# Autodesk Inventor assembly: Protochip
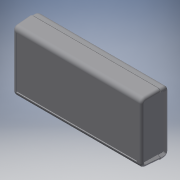
[picture p0: Inventor's stored thumbnail of the model, 180x180]
Saved by Autodesk Inventor 2016 (Build 200138000, 138)
## iProperties
Created: 2011-06-17
Part Number: Protochip
Document SubType Name: Assembly
Designer: David
Title: E:\Eng\Customer Service\Drawings\1593\STEP\1593Y\1593Y Assembly.stp
Author: lwalsh
Sending System: Autodesk Inventor 2011
Preprocessor: Autodesk Inventor 2011
## Documents named in this file (6)
- C:\Users\David\Documents\GitHub\protochip\casing\Protochip.iam
- C:\Users\David\Downloads\1593Y\1593Y Bottom.ipt
- C:\Users\David\Downloads\1593Y\1593Y Top.ipt
- C:\Users\David\Downloads\1593Y\1593Y Battery Cover.ipt
- C:\Users\David\Downloads\1593Y\1593Y Endplate.ipt
- C:\Users\David\Documents\GitHub\protochip\casing\Cheapstat.ipt
## Components (5 placed, 5 different names)
1. 1593Y Bottom:1 — Mate:2
2. 1593Y Top:1
3. 1593Y Battery Cover:1
4. 1593Y Endplate:1 — Mate:1
5. Cheapstat:1 — Mate:1, Mate:2
## Relationships (2: Mate 2)
- Mate:1: 1593Y Endplate:1 ↔ Cheapstat:1
- Mate:2: 1593Y Bottom:1 ↔ Cheapstat:1
